# Autodesk Inventor assembly: Jointed-arm robot
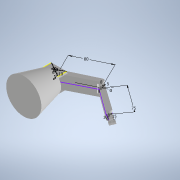
[picture p0: Inventor's stored thumbnail of the model, 180x180]
Saved by Autodesk Inventor 2020 (Build 240168000, 168)
## iProperties
Created: 2020-12-23
Part Number: Jointed-arm robot
Document SubType Name: Assembly
Designer: frost
Author: frost
## Documents named in this file (6)
- C:\Users\frost\OneDrive\Desktop\Intro to Robotics (1)\Jointed-arm robot.iam
- C:\Users\frost\OneDrive\Desktop\Intro to Robotics (1)\base.ipt
- C:\Users\frost\OneDrive\Desktop\Intro to Robotics (1)\shoulder swivel.ipt
- C:\Users\frost\OneDrive\Desktop\Intro to Robotics (1)\Elbow extension.ipt
- C:\Users\frost\OneDrive\Desktop\Intro to Robotics (1)\Pitch and Yaw.ipt
- C:\Users\frost\OneDrive\Desktop\Intro to Robotics (1)\Gripper.ipt
## Components (5 placed, 5 different names)
1. base:1 — Insert:1
2. shoulder swivel:1 — Insert:1, Insert:2
3. Elbow extension:1 — Insert:2, Insert:3
4. Pitch and Yaw:1 — Insert:3, Insert:4
5. Gripper:1 — Insert:4
## Relationships (4: Insert 4)
- Insert:1: base:1 ↔ shoulder swivel:1
- Insert:2: shoulder swivel:1 ↔ Elbow extension:1
- Insert:3: Elbow extension:1 ↔ Pitch and Yaw:1
- Insert:4: Pitch and Yaw:1 ↔ Gripper:1
